# Autodesk Inventor assembly: ASY MSC 300.1 RIGHT BOARD
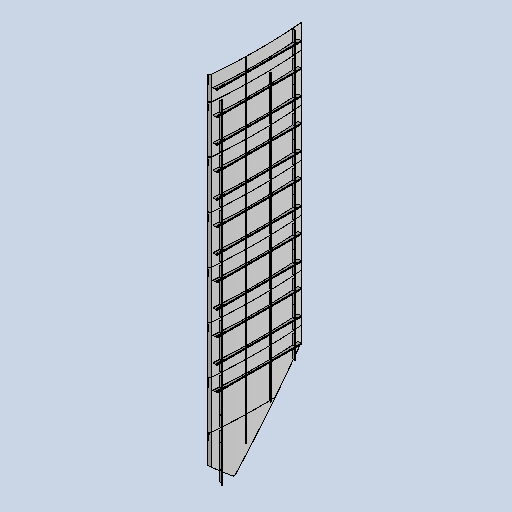
[picture p0: Inventor's stored thumbnail of the model, 512x512]
Saved by Autodesk Inventor 2025 (Build 290162010, 162A)
## iProperties
Created: 2024-07-22
Part Number: ASY MSC 300.1 RIGHT BOARD
Document SubType Name: Assembly
Designer: pokla
Stock Number: ASY МОО 300.1 правый борт
Mass: 330127 g
Surface Area: 285167 cm^2
Volume: 41265.8 cm^3
Density: 8 g/cm^3
Author: pokla
## Documents named in this file (10)
- C:\Users\pokla\Documents\Inventor\Отстойник осветлитель\Manturovo_Se-clar-Gleb\ASY MSC 300.1 RIGHT BOARD.iam
- C:\Users\pokla\Documents\Inventor\Отстойник осветлитель\Manturovo_Se-clar-Gleb\MSC 305 RIB BOARD.ipt
- C:\Users\pokla\Documents\Inventor\Отстойник осветлитель\Manturovo_Se-clar-Gleb\MSC 302 SHEET BOARD MAIN.ipt
- C:\Users\pokla\Documents\Inventor\Отстойник осветлитель\Manturovo_Se-clar-Gleb\MSC 301 SHEET LEFT-RIGHT BOARD HIP.ipt
- C:\Users\pokla\Documents\Inventor\Отстойник осветлитель\Manturovo_Se-clar-Gleb\MSC 303 SHEET RIGHT BOARD WITHERS.ipt
- C:\Users\pokla\Documents\Inventor\Отстойник осветлитель\Manturovo_Se-clar-Gleb\MSC 306 stringer BOARD  #.ipt
- C:\Users\pokla\Documents\Inventor\Отстойник осветлитель\Manturovo_Se-clar-Gleb\MSC 307 stringer BOARD  ##.ipt
- C:\Users\pokla\Documents\Inventor\Отстойник осветлитель\Manturovo_Se-clar-Gleb\MSC 304 SHEET RIGHT BOARD FACE.ipt
- C:\Users\pokla\Documents\Inventor\Отстойник осветлитель\Manturovo_Se-clar-Gleb\MSC 308 stringer BOARD  ###.ipt
- C:\Users\pokla\Documents\Inventor\Отстойник осветлитель\Manturovo_Se-clar-Gleb\MSC 309 stringer BOARD  ####.ipt
## Components (46 placed, 9 different names)
1. MSC 301 SHEET LEFT-RIGHT BOARD HIP.ipt:1 — Flush:2, Flush:3, Flush:4, Rigid:1, Tangent:1, Mate:1
2. MSC 302 SHEET BOARD MAIN.ipt:1 — Rigid:1, Rigid:2, Flush:5
3. MSC 302 SHEET BOARD MAIN.ipt:2 — Rigid:2, Rigid:3
4. MSC 302 SHEET BOARD MAIN.ipt:3 — Rigid:3, Rigid:4
5. MSC 302 SHEET BOARD MAIN.ipt:4 — Rigid:4, Rigid:5
6. MSC 302 SHEET BOARD MAIN.ipt:5 — Rigid:5, Rigid:19
7. MSC 303 SHEET RIGHT BOARD WITHERS.ipt:1 — Rigid:19, Rigid:20
8. MSC 304 SHEET RIGHT BOARD FACE.ipt:1 — Rigid:20
9. MSC 305 RIB BOARD.ipt:1 — Rigid:18, Tangent:1, Mate:1
10. MSC 305 RIB BOARD.ipt:2 — Rigid:12, Rigid:15, Rigid:16, Rigid:17
11. MSC 305 RIB BOARD.ipt:3 — Rigid:13
12. MSC 306 stringer BOARD  #.ipt:1 — Rigid:6, Rigid:12, Rigid:18
13. MSC 307 stringer BOARD  ##.ipt:1 — Rigid:7, Rigid:16, Flush:5
14. MSC 308 stringer BOARD  ###.ipt:1 — Rigid:8, Rigid:9
15. MSC 309 stringer BOARD  ####.ipt:1 — Rigid:10, Rigid:11
16. MSC 309 stringer BOARD  ####.ipt:2 — Rigid:10, Rigid:15
17. MSC 308 stringer BOARD  ###.ipt:2 — Rigid:8, Rigid:17
18. MSC 305 RIB BOARD.ipt:4 — Rigid:14
19. MSC 305 RIB BOARD.ipt:5
20. MSC 305 RIB BOARD.ipt:6
21. MSC 305 RIB BOARD.ipt:7
22. MSC 305 RIB BOARD.ipt:8
23. MSC 305 RIB BOARD.ipt:9
24. MSC 305 RIB BOARD.ipt:10
25. MSC 305 RIB BOARD.ipt:11
26. MSC 305 RIB BOARD.ipt:12
27. MSC 306 stringer BOARD  #.ipt:2 — Rigid:6, Rigid:13, Rigid:14
28. MSC 307 stringer BOARD  ##.ipt:2 — Rigid:7
29. MSC 308 stringer BOARD  ###.ipt:3 — Rigid:9
30. MSC 309 stringer BOARD  ####.ipt:3 — Rigid:11
31. MSC 306 stringer BOARD  #.ipt:3
32. MSC 307 stringer BOARD  ##.ipt:3
33. MSC 308 stringer BOARD  ###.ipt:4
34. MSC 309 stringer BOARD  ####.ipt:4
35. MSC 306 stringer BOARD  #.ipt:4
36. MSC 307 stringer BOARD  ##.ipt:4
37. MSC 308 stringer BOARD  ###.ipt:5
38. MSC 309 stringer BOARD  ####.ipt:5
39. MSC 306 stringer BOARD  #.ipt:5
40. MSC 307 stringer BOARD  ##.ipt:5
41. MSC 308 stringer BOARD  ###.ipt:6
42. MSC 309 stringer BOARD  ####.ipt:6
43. MSC 306 stringer BOARD  #.ipt:6
44. MSC 307 stringer BOARD  ##.ipt:6
45. MSC 308 stringer BOARD  ###.ipt:7
46. MSC 309 stringer BOARD  ####.ipt:7
## Component patterns: (9 elements, first: MSC 305 RIB BOARD.ipt:4), (5 elements, first: MSC 306 stringer BOARD  #.ipt:2 + MSC 307 stringer BOARD  ##.ipt:2 + MSC 308 stringer BOARD  ###.ipt:3 + MSC 309 stringer BOARD  ####.ipt:3)
## Relationships (26: WeldJoint 20, Flush 4, Tangent 1, Mate 1)
- Flush:2: MSC 301 SHEET LEFT-RIGHT BOARD HIP.ipt:1
- Flush:3: MSC 301 SHEET LEFT-RIGHT BOARD HIP.ipt:1
- Flush:4: MSC 301 SHEET LEFT-RIGHT BOARD HIP.ipt:1
- Rigid:1 [WeldJoint]: MSC 301 SHEET LEFT-RIGHT BOARD HIP.ipt:1 ↔ MSC 302 SHEET BOARD MAIN.ipt:1
- Rigid:2 [WeldJoint]: MSC 302 SHEET BOARD MAIN.ipt:1 ↔ MSC 302 SHEET BOARD MAIN.ipt:2
- Rigid:3 [WeldJoint]: MSC 302 SHEET BOARD MAIN.ipt:2 ↔ MSC 302 SHEET BOARD MAIN.ipt:3
- Rigid:4 [WeldJoint]: MSC 302 SHEET BOARD MAIN.ipt:3 ↔ MSC 302 SHEET BOARD MAIN.ipt:4
- Rigid:5 [WeldJoint]: MSC 302 SHEET BOARD MAIN.ipt:4 ↔ MSC 302 SHEET BOARD MAIN.ipt:5
- Rigid:6 [WeldJoint]: MSC 306 stringer BOARD  #.ipt:1 ↔ MSC 306 stringer BOARD  #.ipt:2
- Rigid:7 [WeldJoint]: MSC 307 stringer BOARD  ##.ipt:1 ↔ MSC 307 stringer BOARD  ##.ipt:2
- Rigid:8 [WeldJoint]: MSC 308 stringer BOARD  ###.ipt:1 ↔ MSC 308 stringer BOARD  ###.ipt:2
- Rigid:9 [WeldJoint]: MSC 308 stringer BOARD  ###.ipt:1 ↔ MSC 308 stringer BOARD  ###.ipt:3
- Rigid:10 [WeldJoint]: MSC 309 stringer BOARD  ####.ipt:1 ↔ MSC 309 stringer BOARD  ####.ipt:2
- Rigid:11 [WeldJoint]: MSC 309 stringer BOARD  ####.ipt:1 ↔ MSC 309 stringer BOARD  ####.ipt:3
- Rigid:12 [WeldJoint] (2 mm): MSC 305 RIB BOARD.ipt:2 ↔ MSC 306 stringer BOARD  #.ipt:1
- Rigid:13 [WeldJoint] (2 mm): MSC 305 RIB BOARD.ipt:3 ↔ MSC 306 stringer BOARD  #.ipt:2
- Rigid:14 [WeldJoint] (2 mm): MSC 305 RIB BOARD.ipt:4 ↔ MSC 306 stringer BOARD  #.ipt:2
- Rigid:15 [WeldJoint] (2 mm): MSC 305 RIB BOARD.ipt:2 ↔ MSC 309 stringer BOARD  ####.ipt:2
- Rigid:16 [WeldJoint] (2 mm): MSC 305 RIB BOARD.ipt:2 ↔ MSC 307 stringer BOARD  ##.ipt:1
- Rigid:17 [WeldJoint] (2 mm): MSC 305 RIB BOARD.ipt:2 ↔ MSC 308 stringer BOARD  ###.ipt:2
- Rigid:18 [WeldJoint] (2 mm): MSC 305 RIB BOARD.ipt:1 ↔ MSC 306 stringer BOARD  #.ipt:1
- Rigid:19 [WeldJoint]: MSC 302 SHEET BOARD MAIN.ipt:5 ↔ MSC 303 SHEET RIGHT BOARD WITHERS.ipt:1
- Rigid:20 [WeldJoint]: MSC 303 SHEET RIGHT BOARD WITHERS.ipt:1 ↔ MSC 304 SHEET RIGHT BOARD FACE.ipt:1
- Flush:5: MSC 302 SHEET BOARD MAIN.ipt:1 ↔ MSC 307 stringer BOARD  ##.ipt:1
- Tangent:1: MSC 301 SHEET LEFT-RIGHT BOARD HIP.ipt:1 ↔ MSC 305 RIB BOARD.ipt:1
- Mate:1 (75 mm): MSC 301 SHEET LEFT-RIGHT BOARD HIP.ipt:1 ↔ MSC 305 RIB BOARD.ipt:1
